# Autodesk Inventor assembly: keywell
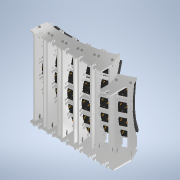
[picture p0: Inventor's stored thumbnail of the model, 180x180]
Saved by Autodesk Inventor 2020.1 (Build 241239000, 239)
## iProperties
Created: 2019-07-06
Part Number: keywell
Document SubType Name: Assembly
Designer: Thibault
Mass: 341.563 g
Surface Area: 1996.11 cm^2
Volume: 92.7912 cm^3
Density: 3.68098 g/cm^3
Author: Thibault
## Documents named in this file (13)
- C:\Users\Thibault Polge\Documents\Habilis\mech\keywell.iam
- C:\Users\Thibault Polge\Documents\Habilis\mech\switchplate\switchplate-1.iam
- C:\Users\Thibault Polge\Documents\Habilis\mech\switchplate.iam
- C:\Users\Thibault Polge\Documents\Habilis\mech\switchplate\switchplate-2.iam
- C:\Users\Thibault Polge\Documents\Habilis\mech\switchplate\switchplate-3.iam
- C:\Users\Thibault Polge\Documents\Habilis\mech\switchplate\switchplate-4.iam
- C:\Users\Thibault Polge\Documents\Habilis\mech\switchplate\switchplate-5.iam
- C:\Users\Thibault Polge\Documents\Habilis\mech\switchplate\switchplate-6.iam
- C:\Users\Thibault Polge\Documents\Habilis\mech\keywell_support\keywell_support-back.ipt
- C:\Users\Thibault Polge\Documents\Habilis\mech\keywell_support.ipt
- C:\Users\Thibault Polge\Documents\Habilis\mech\keywell_support\keywell_support-front.ipt
- C:\Users\Thibault Polge\Documents\Habilis\mech\keywell_support\keywell_support-front-r6.ipt
- C:\Users\Thibault Polge\Documents\Inventor\Content Center Files\R2020\fr-FR\BS 4168(1)\BS 4168 - M1,6 x 8(1).ipt
## Components (33 placed, 10 different names)
1. keywell_support-back:1 — Affleurement:1, Affleurement:3, Affleurement:4, Affleurement:5, Affleurement:6, Affleurement:9, Logement:13, Logement:14, Logement:15, Logement:16, Logement:17, Logement:18, Logement:19, Logement:20, Logement:21, Logement:22, Logement:23, Logement:24, Placage:1, Placage:2, Placage:3, Placage:4, Placage:5, Placage:6, Placage:7, Placage:8, Placage:9, Placage:10, Placage:11, Placage:12
2. switchplate-1:1 [sub-assembly] — Affleurement:1, Affleurement:7, Placage:1, Placage:12
3. switchplate-2:2 [sub-assembly] — Affleurement:9, Placage:2, Placage:11
4. switchplate-3:3 [sub-assembly] — Affleurement:3, Placage:3, Placage:10
5. switchplate-4:4 [sub-assembly] — Affleurement:4, Placage:4, Placage:9
6. switchplate-5:5 [sub-assembly] — Affleurement:5, Placage:5, Placage:8
7. switchplate-6:6 [sub-assembly] — Affleurement:6, Placage:6, Placage:7, Affleurement:10, Placage:13, Placage:14
8. keywell_support-front:2 — Affleurement:7, Logement:1, Logement:2, Logement:3, Logement:4, Logement:5, Logement:6, Logement:7, Logement:8, Logement:9, Logement:10
9. keywell_support-front-r6:3 — Logement:11, Logement:12, Affleurement:10, Placage:13, Placage:14
10. BS 4168 : Pièce 1 Vis cylindrique à six pans creux - Métrique M1,6 x 8:1 — Logement:1
11. BS 4168 : Pièce 1 Vis cylindrique à six pans creux - Métrique M1,6 x 8:2 — Logement:2
12. BS 4168 : Pièce 1 Vis cylindrique à six pans creux - Métrique M1,6 x 8:3 — Logement:3
13. BS 4168 : Pièce 1 Vis cylindrique à six pans creux - Métrique M1,6 x 8:4 — Logement:4
14. BS 4168 : Pièce 1 Vis cylindrique à six pans creux - Métrique M1,6 x 8:5 — Logement:5
15. BS 4168 : Pièce 1 Vis cylindrique à six pans creux - Métrique M1,6 x 8:6 — Logement:6
16. BS 4168 : Pièce 1 Vis cylindrique à six pans creux - Métrique M1,6 x 8:7 — Logement:7
17. BS 4168 : Pièce 1 Vis cylindrique à six pans creux - Métrique M1,6 x 8:8 — Logement:8
18. BS 4168 : Pièce 1 Vis cylindrique à six pans creux - Métrique M1,6 x 8:9 — Logement:9
19. BS 4168 : Pièce 1 Vis cylindrique à six pans creux - Métrique M1,6 x 8:10 — Logement:10
20. BS 4168 : Pièce 1 Vis cylindrique à six pans creux - Métrique M1,6 x 8:11 — Logement:11
21. BS 4168 : Pièce 1 Vis cylindrique à six pans creux - Métrique M1,6 x 8:12 — Logement:12
22. BS 4168 : Pièce 1 Vis cylindrique à six pans creux - Métrique M1,6 x 8:13 — Logement:13
23. BS 4168 : Pièce 1 Vis cylindrique à six pans creux - Métrique M1,6 x 8:14 — Logement:14
24. BS 4168 : Pièce 1 Vis cylindrique à six pans creux - Métrique M1,6 x 8:15 — Logement:15
25. BS 4168 : Pièce 1 Vis cylindrique à six pans creux - Métrique M1,6 x 8:16 — Logement:16
26. BS 4168 : Pièce 1 Vis cylindrique à six pans creux - Métrique M1,6 x 8:17 — Logement:17
27. BS 4168 : Pièce 1 Vis cylindrique à six pans creux - Métrique M1,6 x 8:18 — Logement:18
28. BS 4168 : Pièce 1 Vis cylindrique à six pans creux - Métrique M1,6 x 8:19 — Logement:19
29. BS 4168 : Pièce 1 Vis cylindrique à six pans creux - Métrique M1,6 x 8:20 — Logement:20
30. BS 4168 : Pièce 1 Vis cylindrique à six pans creux - Métrique M1,6 x 8:21 — Logement:21
31. BS 4168 : Pièce 1 Vis cylindrique à six pans creux - Métrique M1,6 x 8:22 — Logement:22
32. BS 4168 : Pièce 1 Vis cylindrique à six pans creux - Métrique M1,6 x 8:23 — Logement:23
33. BS 4168 : Pièce 1 Vis cylindrique à six pans creux - Métrique M1,6 x 8:24 — Logement:24
## Relationships (46: Insert 24, Mate 14, Flush 8)
- Affleurement:1 [Flush]: keywell_support-back:1 ↔ switchplate-1:1
- Affleurement:3 [Flush]: keywell_support-back:1 ↔ switchplate-3:3
- Affleurement:4 [Flush]: keywell_support-back:1 ↔ switchplate-4:4
- Affleurement:5 [Flush]: keywell_support-back:1 ↔ switchplate-5:5
- Affleurement:6 [Flush]: keywell_support-back:1 ↔ switchplate-6:6
- Affleurement:7 [Flush]: switchplate-1:1 ↔ keywell_support-front:2
- Affleurement:9 [Flush]: keywell_support-back:1 ↔ switchplate-2:2
- Logement:1 [Insert]: keywell_support-front:2 ↔ BS 4168 : Pièce 1 Vis cylindrique à six pans creux - Métrique M1,6 x 8:1
- Logement:2 [Insert]: keywell_support-front:2 ↔ BS 4168 : Pièce 1 Vis cylindrique à six pans creux - Métrique M1,6 x 8:2
- Logement:3 [Insert]: keywell_support-front:2 ↔ BS 4168 : Pièce 1 Vis cylindrique à six pans creux - Métrique M1,6 x 8:3
- Logement:4 [Insert]: keywell_support-front:2 ↔ BS 4168 : Pièce 1 Vis cylindrique à six pans creux - Métrique M1,6 x 8:4
- Logement:5 [Insert]: keywell_support-front:2 ↔ BS 4168 : Pièce 1 Vis cylindrique à six pans creux - Métrique M1,6 x 8:5
- Logement:6 [Insert]: keywell_support-front:2 ↔ BS 4168 : Pièce 1 Vis cylindrique à six pans creux - Métrique M1,6 x 8:6
- Logement:7 [Insert]: keywell_support-front:2 ↔ BS 4168 : Pièce 1 Vis cylindrique à six pans creux - Métrique M1,6 x 8:7
- Logement:8 [Insert]: keywell_support-front:2 ↔ BS 4168 : Pièce 1 Vis cylindrique à six pans creux - Métrique M1,6 x 8:8
- Logement:9 [Insert]: keywell_support-front:2 ↔ BS 4168 : Pièce 1 Vis cylindrique à six pans creux - Métrique M1,6 x 8:9
- Logement:10 [Insert]: keywell_support-front:2 ↔ BS 4168 : Pièce 1 Vis cylindrique à six pans creux - Métrique M1,6 x 8:10
- Logement:11 [Insert]: keywell_support-front-r6:3 ↔ BS 4168 : Pièce 1 Vis cylindrique à six pans creux - Métrique M1,6 x 8:11
- Logement:12 [Insert]: keywell_support-front-r6:3 ↔ BS 4168 : Pièce 1 Vis cylindrique à six pans creux - Métrique M1,6 x 8:12
- Logement:13 [Insert]: keywell_support-back:1 ↔ BS 4168 : Pièce 1 Vis cylindrique à six pans creux - Métrique M1,6 x 8:13
- Logement:14 [Insert]: keywell_support-back:1 ↔ BS 4168 : Pièce 1 Vis cylindrique à six pans creux - Métrique M1,6 x 8:14
- Logement:15 [Insert]: keywell_support-back:1 ↔ BS 4168 : Pièce 1 Vis cylindrique à six pans creux - Métrique M1,6 x 8:15
- Logement:16 [Insert]: keywell_support-back:1 ↔ BS 4168 : Pièce 1 Vis cylindrique à six pans creux - Métrique M1,6 x 8:16
- Logement:17 [Insert]: keywell_support-back:1 ↔ BS 4168 : Pièce 1 Vis cylindrique à six pans creux - Métrique M1,6 x 8:17
- Logement:18 [Insert]: keywell_support-back:1 ↔ BS 4168 : Pièce 1 Vis cylindrique à six pans creux - Métrique M1,6 x 8:18
- Logement:19 [Insert]: keywell_support-back:1 ↔ BS 4168 : Pièce 1 Vis cylindrique à six pans creux - Métrique M1,6 x 8:19
- Logement:20 [Insert]: keywell_support-back:1 ↔ BS 4168 : Pièce 1 Vis cylindrique à six pans creux - Métrique M1,6 x 8:20
- Logement:21 [Insert]: keywell_support-back:1 ↔ BS 4168 : Pièce 1 Vis cylindrique à six pans creux - Métrique M1,6 x 8:21
- Logement:22 [Insert]: keywell_support-back:1 ↔ BS 4168 : Pièce 1 Vis cylindrique à six pans creux - Métrique M1,6 x 8:22
- Logement:23 [Insert]: keywell_support-back:1 ↔ BS 4168 : Pièce 1 Vis cylindrique à six pans creux - Métrique M1,6 x 8:23
- Logement:24 [Insert]: keywell_support-back:1 ↔ BS 4168 : Pièce 1 Vis cylindrique à six pans creux - Métrique M1,6 x 8:24
- Placage:1 [Mate]: keywell_support-back:1 ↔ switchplate-1:1
- Placage:2 [Mate]: keywell_support-back:1 ↔ switchplate-2:2
- Placage:3 [Mate]: keywell_support-back:1 ↔ switchplate-3:3
- Placage:4 [Mate]: keywell_support-back:1 ↔ switchplate-4:4
- Placage:5 [Mate]: keywell_support-back:1 ↔ switchplate-5:5
- Placage:6 [Mate]: keywell_support-back:1 ↔ switchplate-6:6
- Placage:7 [Mate]: keywell_support-back:1 ↔ switchplate-6:6
- Placage:8 [Mate]: keywell_support-back:1 ↔ switchplate-5:5
- Placage:9 [Mate]: keywell_support-back:1 ↔ switchplate-4:4
- Placage:10 [Mate]: keywell_support-back:1 ↔ switchplate-3:3
- Placage:11 [Mate]: keywell_support-back:1 ↔ switchplate-2:2
- Placage:12 [Mate]: keywell_support-back:1 ↔ switchplate-1:1
- Affleurement:10 [Flush]: switchplate-6:6 ↔ keywell_support-front-r6:3
- Placage:13 [Mate]: switchplate-6:6 ↔ keywell_support-front-r6:3
- Placage:14 [Mate]: switchplate-6:6 ↔ keywell_support-front-r6:3
